# Autodesk Inventor assembly: BandeV2
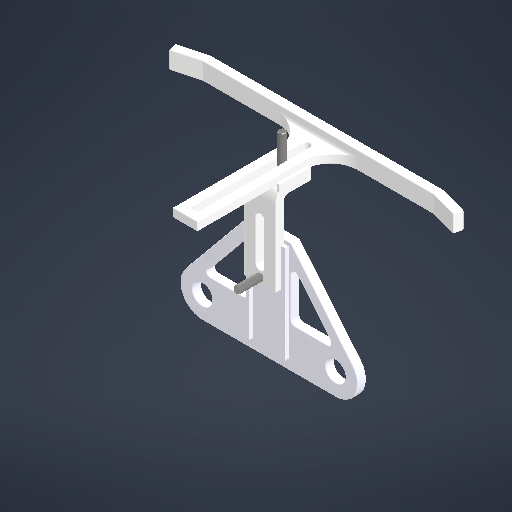
[picture p0: Inventor's stored thumbnail of the model, 512x512]
Saved by Autodesk Inventor 2026.3 (Build 303398000, 398)
## iProperties
Created: 2026-06-25
Part Number: BandeV2
Document SubType Name: Assembly
Designer: frede
Author: frede
## Documents named in this file (5)
- E:\Git\AppliedAutomationProject\CAD\bander\BandeV2.iam
- E:\Git\AppliedAutomationProject\CAD\bander\BandeV2Base.ipt
- D:\OneDrive\Dokumenter\Inventor\Content Center Files\R2026\en-US\BS EN ISO 4017\BS EN ISO 4017 - M4 x 20BS EN.ipt
- E:\Git\AppliedAutomationProject\CAD\bander\BandeV2Joint2.ipt
- E:\Git\AppliedAutomationProject\CAD\bander\BandeV2Joint3.ipt
## Components (5 placed, 4 different names)
1. BandeV2Base:1 — Insert:1, Angle:1, Flush:1, Mate:1
2. BS EN ISO 4017 - Metric M4 x 20:1 — Insert:1, Angle:1
3. BandeV2Joint2:1 — Flush:1, Mate:1, Insert:2, Angle:2, Flush:2, Mate:2
4. BS EN ISO 4017 - Metric M4 x 20:2 — Insert:2, Angle:2
5. BandeV2Joint3:1 — Flush:2, Mate:2
## Relationships (8: Insert 2, Angle 2, Flush 2, Mate 2)
- Insert:1: BandeV2Base:1 ↔ BS EN ISO 4017 - Metric M4 x 20:1
- Angle:1 (0 deg): BandeV2Base:1 ↔ BS EN ISO 4017 - Metric M4 x 20:1
- Flush:1: BandeV2Base:1 ↔ BandeV2Joint2:1
- Mate:1 (0.1 mm): BandeV2Base:1 ↔ BandeV2Joint2:1
- Insert:2: BandeV2Joint2:1 ↔ BS EN ISO 4017 - Metric M4 x 20:2
- Angle:2 (0 deg): BandeV2Joint2:1 ↔ BS EN ISO 4017 - Metric M4 x 20:2
- Flush:2: BandeV2Joint2:1 ↔ BandeV2Joint3:1
- Mate:2 (0.1 mm): BandeV2Joint2:1 ↔ BandeV2Joint3:1
